# Autodesk Inventor assembly: Sliders block
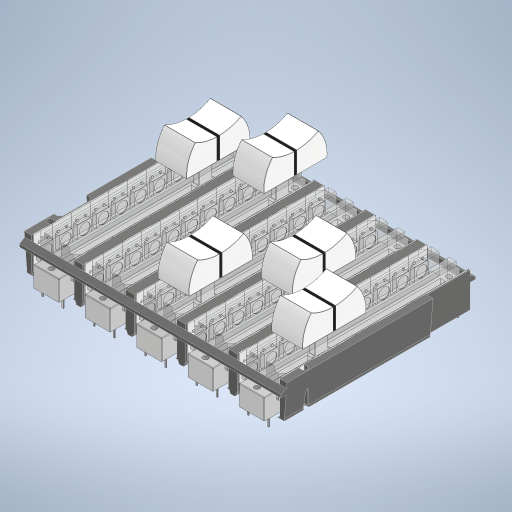
[picture p0: Inventor's stored thumbnail of the model, 512x512]
Saved by Autodesk Inventor 2023 (Build 270158000, 158)
## iProperties
Created: 2024-03-26
Part Number: Sliders block
Document SubType Name: Assembly
Designer: noname
Author: noname
## Documents named in this file (3)
- C:\Users\noname\Documents\GitHub\AudMix\3dModels\Sliders block.iam
- C:\Users\noname\Documents\GitHub\AudMix\3dModels\Slider with leds.iam
- C:\Users\noname\Documents\GitHub\AudMix\3dModels\Brackets.ipt
## Components (6 placed, 2 different names)
1. Slider with leds:1 [sub-assembly] — Mate:5, Mate:6, Flush:5
2. Slider with leds:2 [sub-assembly] — Mate:3, Mate:8, Flush:3
3. Slider with leds:3 [sub-assembly] — Mate:2, Mate:9, Flush:2
4. Slider with leds:4 [sub-assembly] — Mate:1, Mate:10, Flush:1
5. Slider with leds:5 [sub-assembly] — Mate:4, Mate:7, Flush:4
6. Brackets:1 — Mate:1, Mate:2, Mate:3, Mate:4, Mate:5, Mate:6, Mate:7, Mate:8, Mate:9, Mate:10, Flush:1, Flush:2, Flush:3, Flush:4, Flush:5
## Relationships (15: Mate 10, Flush 5)
- Mate:1: Slider with leds:4 ↔ Brackets:1
- Mate:2: Slider with leds:3 ↔ Brackets:1
- Mate:3: Slider with leds:2 ↔ Brackets:1
- Mate:4: Slider with leds:5 ↔ Brackets:1
- Mate:5: Slider with leds:1 ↔ Brackets:1
- Mate:6: Slider with leds:1 ↔ Brackets:1
- Mate:7: Slider with leds:5 ↔ Brackets:1
- Mate:8: Slider with leds:2 ↔ Brackets:1
- Mate:9: Slider with leds:3 ↔ Brackets:1
- Mate:10: Slider with leds:4 ↔ Brackets:1
- Flush:1: Slider with leds:4 ↔ Brackets:1
- Flush:2: Slider with leds:3 ↔ Brackets:1
- Flush:3: Slider with leds:2 ↔ Brackets:1
- Flush:4: Slider with leds:5 ↔ Brackets:1
- Flush:5: Slider with leds:1 ↔ Brackets:1
